# Autodesk Inventor assembly: BG001_trajan20_21
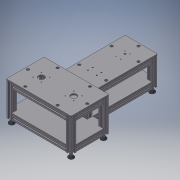
[picture p0: Inventor's stored thumbnail of the model, 180x180]
Saved by Autodesk Inventor 2022.2 (Build 262287000, 287)
## iProperties
Company: HTBLA Kaindorf
RuleStatus: InUse
Created: 2022-08-03
Part Number: BG001_trajan20_21
Project: Zeichenmaschine_v2
Material: Generisch
Description: Gerüst mit Platten
Document SubType Name: Assembly
Designer: trajan20
AfterDocNew0: iProperties-Editor_aufrufen
Author: jan
Keywords: 2021
## Documents named in this file (5)
- C:\Users\jan\Documents\DrawMachine\DrawMachineConstruction\Projekt\Zeichenmaschine_v2\BG001_trajan20_21_Zeichenmaschine_v2_Gerüst mit Platten.iam
- C:\Users\jan\Documents\DrawMachine\DrawMachineConstruction\Projekt\Zeichenmaschine_v2\Gerüst_v2.iam
- C:\Users\jan\Documents\DrawMachine\DrawMachineConstruction\Projekt\Zeichenmaschine_v2\BT001_trajan20_21_Zeichenmaschine_v2_Platte Stepper Motoren.ipt
- C:\Users\jan\Documents\DrawMachine\DrawMachineConstruction\Projekt\Zeichenmaschine_v2\BT002_trajan20_21_Zeichenmaschine_v2_Platte Getriebemotor.ipt
- C:\Users\jan\Documents\DrawMachine\DrawMachineConstruction\Projekt\Zeichenmaschine_v2\BT003_trajan20_21_Zeichenmaschine_v2_Platte unten.ipt
## Components (4 placed, 4 different names)
1. Gerüst_v2:1 [sub-assembly] — Passend:1, Fluchtend:1, Fluchtend:2, Passend:2, Fluchtend:3, Fluchtend:4, Passend:3, Fluchtend:5, Fluchtend:6
2. BT001_trajan20_21_Zeichenmaschine_v2_Platte Stepper Motoren:1 — Passend:1, Fluchtend:1, Fluchtend:2
3. BT002_trajan20_21_Zeichenmaschine_v2_Platte Getriebemotor:1 — Passend:2, Fluchtend:3, Fluchtend:4
4. BT003_trajan20_21_Zeichenmaschine_v2_Platte unten:1 — Passend:3, Fluchtend:5, Fluchtend:6
## Relationships (9: Flush 6, Mate 3)
- Passend:1 [Mate]: Gerüst_v2:1 ↔ BT001_trajan20_21_Zeichenmaschine_v2_Platte Stepper Motoren:1
- Fluchtend:1 [Flush]: Gerüst_v2:1 ↔ BT001_trajan20_21_Zeichenmaschine_v2_Platte Stepper Motoren:1
- Fluchtend:2 [Flush]: Gerüst_v2:1 ↔ BT001_trajan20_21_Zeichenmaschine_v2_Platte Stepper Motoren:1
- Passend:2 [Mate]: Gerüst_v2:1 ↔ BT002_trajan20_21_Zeichenmaschine_v2_Platte Getriebemotor:1
- Fluchtend:3 [Flush]: Gerüst_v2:1 ↔ BT002_trajan20_21_Zeichenmaschine_v2_Platte Getriebemotor:1
- Fluchtend:4 [Flush]: Gerüst_v2:1 ↔ BT002_trajan20_21_Zeichenmaschine_v2_Platte Getriebemotor:1
- Passend:3 [Mate]: Gerüst_v2:1 ↔ BT003_trajan20_21_Zeichenmaschine_v2_Platte unten:1
- Fluchtend:5 [Flush]: Gerüst_v2:1 ↔ BT003_trajan20_21_Zeichenmaschine_v2_Platte unten:1
- Fluchtend:6 [Flush]: Gerüst_v2:1 ↔ BT003_trajan20_21_Zeichenmaschine_v2_Platte unten:1
